# Autodesk Inventor assembly: R-H v20
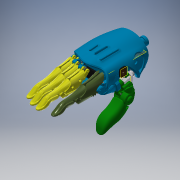
[picture p0: Inventor's stored thumbnail of the model, 180x180]
Saved by Autodesk Inventor 2018.2 (Build 222227000, 227)
## iProperties
Created: 2017-09-22
Part Number: R-H v20
Material: 一般
Document SubType Name: Assembly
Designer: sktom
Author: sktom
## Documents named in this file (41)
- D:\CloudStrage\OneDrive\CADMech\HbSizeMMech\UnitHand\Unit_MR-H\Unit_MR-H.iam
- D:\CloudStrage\OneDrive\CADMech\HbSizeMMech\UnitHand\Unit_MR-H\Parts_MR-H\MR-H-01.ipt
- D:\CloudStrage\OneDrive\CADMech\HbSizeMMech\UnitHand\Unit_MR-H\Parts_MR-H\MR-H-02.ipt
- D:\CloudStrage\OneDrive\CADMech\HbSizeMMech\UnitHand\Unit_MR-H\Parts_MR-H\MR-H-03.ipt
- D:\CloudStrage\OneDrive\CADMech\HbSizeMMech\UnitHand\Unit_MR-H\Parts_MR-H\MR-H-04.ipt
- D:\CloudStrage\OneDrive\CADMech\HbSizeMMech\UnitHand\Unit_MR-H\Unit_MR-I\Unit_MR-I .iam
- D:\CloudStrage\OneDrive\CADMech\HbSizeMMech\UnitHand\Unit_MR-H\Unit_MR-O\Unit_MR-O.iam
- D:\CloudStrage\OneDrive\CADMech\HbSizeMMech\UnitHand\Unit_MR-H\Parts_MR-H\MR-H-05.ipt
- D:\CloudStrage\OneDrive\CADMech\HbSizeMMech\UnitHand\Unit_MR-H\Parts_MR-H\MR-H-06.ipt
- D:\CloudStrage\OneDrive\CADMech\HbSizeMMech\UnitHand\Unit_MR-H\Parts_MR-H\MR-H-07.ipt
- D:\CloudStrage\OneDrive\CADMech\HbSizeMMech\UnitHand\Unit_MR-H\Parts_MR-H\MR-H-08.ipt
- D:\CloudStrage\OneDrive\CADMech\HbSizeMMech\UnitHand\Unit_MR-H\Parts_MR-H\MR-H-15.ipt
- D:\CloudStrage\OneDrive\CADMech\HbSizeMMech\UnitHand\Unit_MR-H\Parts_MR-H\MR-H-10.ipt
- D:\CloudStrage\OneDrive\CADMech\HbSizeMMech\UnitHand\Unit_MR-H\Parts_MR-H\MR-H-11.ipt
- D:\CloudStrage\OneDrive\CADMech\HbSizeMMech\UnitHand\Unit_MR-H\Parts_MR-H\MR-H-12.ipt
- D:\CloudStrage\OneDrive\CADMech\HbSizeMMech\UnitHand\Unit_MR-H\Parts_MR-H\MR-H-13.ipt
- D:\CloudStrage\OneDrive\CADMech\HbSizeMMech\UnitHand\Unit_MR-H\Parts_MR-H\MR-H-14.ipt
- D:\CloudStrage\OneDrive\CADMech\HbSizeMMech\UnitHand\Unit_MR-H\Unit_MR-T\Unit_MR-T.iam
- D:\CloudStrage\OneDrive\CADMech\HbSizeMMech\UnitHand\Unit_MR-H\Parts_MR-H\Parts_bearing_FL674ZZ.ipt
- D:\CloudStrage\OneDrive\CADMech\HbSizeMMech\UnitHand\Unit_MR-H\Parts_MR-H\Parts_Servo_Micro2BBMG.ipt
- D:\CloudStrage\OneDrive\CADMech\HbSizeMMech\UnitHand\Unit_MR-H\Parts_MR-H\Parts_Servo_HK282A_Hone.ipt
- D:\CloudStrage\OneDrive\CADMech\HbSizeMMech\UnitHand\Unit_MR-H\Parts_MR-H\Parts_Servo_ASV-15MG.ipt
- D:\CloudStrage\OneDrive\CADMech\HbSizeMMech\UnitHand\Unit_MR-H\Parts_MR-H\MR-H-09.ipt
- D:\CloudStrage\OneDrive\CADMech\HbSizeMMech\UnitHand\Unit_MR-H\Parts_MR-H\Circuit_handmainboard.ipt
- D:\CloudStrage\OneDrive\CADMech\HbSizeMMech\UnitHand\Unit_MR-H\Parts_MR-H\Parts_Screw_M1.7_L8.ipt
- D:\CloudStrage\OneDrive\CADMech\HbSizeMMech\UnitHand\Unit_MR-H\Parts_MR-H\Parts_Screw_M2_L8.ipt
- D:\CloudStrage\OneDrive\CADMech\HbSizeMMech\UnitHand\Unit_MR-H\Parts_MR-H\Parts_Screw_M3_L6.ipt
- D:\CloudStrage\OneDrive\CADMech\HbSizeMMech\UnitHand\Unit_MR-H\Parts_MR-H\Parts_Servo_Micro2BBMG_hone.ipt
- D:\CloudStrage\OneDrive\CADMech\HbSizeMMech\UnitHand\Unit_MR-H\Parts_MR-H\Parts_FlatScrew_M2_L6.ipt
- D:\CloudStrage\OneDrive\CADMech\HbSizeMMech\UnitHand\Unit_MR-H\Parts_MR-H\Parts_Shaft_Phi2_L12.ipt
- D:\CloudStrage\OneDrive\CADMech\HbSizeMMech\UnitHand\Unit_MR-H\Parts_MR-H\Parts_MetalCollar_Ph2_L4.5.ipt
- D:\CloudStrage\OneDrive\CADMech\HbSizeMMech\UnitHand\Unit_MR-H\Parts_MR-H\Parts_Washer_M2_Ph4.3_T0.3.ipt
- D:\CloudStrage\OneDrive\CADMech\HbSizeMMech\UnitHand\Unit_MR-H\Parts_MR-H\Parts_Servo_ASV-15MG_Hone.ipt
- D:\CloudStrage\OneDrive\CADMech\HbSizeMMech\UnitHand\Unit_MR-H\Parts_MR-H\Circuit_Controller_Pololu-A-Star-32U4-Micro.ipt
- D:\CloudStrage\OneDrive\CADMech\HbSizeMMech\UnitHand\Unit_MR-H\Parts_MR-H\Circuit_DCDCconverter_OKL-T3-W12N-C.ipt
- D:\CloudStrage\OneDrive\CADMech\HbSizeMMech\UnitHand\Unit_MR-H\Parts_MR-H\Circuit_DCjack_MJ179PH.ipt
- D:\CloudStrage\OneDrive\CADMech\HbSizeMMech\UnitHand\Unit_MR-H\Parts_MR-H\Circuit_Connector_533980371.ipt
- D:\CloudStrage\OneDrive\CADMech\HbSizeMMech\UnitHand\Unit_MR-H\Parts_MR-H\Circuit_Connector_H3-2.ipt
- D:\CloudStrage\OneDrive\CADMech\HbSizeMMech\UnitHand\Unit_MR-H\Parts_MR-H\Circuit_TactSwitch_SKRPACE010.ipt
- D:\CloudStrage\OneDrive\CADMech\HbSizeMMech\UnitHand\Unit_MR-H\Parts_MR-H\Circuit_SlideSwitch_SS-12D00-G5.ipt
- D:\CloudStrage\OneDrive\CADMech\HbSizeMMech\UnitHand\Unit_MR-H\Parts_MR-H\Circuit_PinHeader_PSM-410233-00.ipt
## Components (89 placed, 40 different names)
1. Unit_MR-I [sub-assembly] — メイト:25, 円柱状:15
2. Unit_MR-T:1 [sub-assembly]
3. Unit_MR-O:2 [sub-assembly] — 挿入:42, 円柱状:5, 円柱状:6, メイト:22, 挿入:43
4. Unit_MR-O:4 [sub-assembly] — メイト:24, 円柱状:12, 円柱状:13, 挿入:54, 挿入:55, 挿入:56
5. Unit_MR-O:3 [sub-assembly] — メイト:23, 円柱状:8, 円柱状:9, 挿入:46, 挿入:49, 挿入:50, 挿入:51
6. MR-H-01:1
7. MR-H-02:1 — 挿入:1, 挿入:2, 挿入:13, 挿入:14, 挿入:17, 挿入:18, 挿入:22, 挿入:26, 挿入:32, 挿入:33, 円柱状:5, 円柱状:6, メイト:22, メイト:23, 円柱状:8, 円柱状:9, メイト:24, 円柱状:12, 円柱状:13, メイト:25, 円柱状:15, 挿入:59, 挿入:60, 円柱状:16, 挿入:61, 円柱状:17, 挿入:62, 円柱状:18, 挿入:63, 挿入:64, 挿入:65, 挿入:66, 挿入:67, 円柱状:19, メイト:30
8. MR-H-03:1 — 挿入:26, 挿入:27
9. MR-H-04:1 — 挿入:22, 挿入:23
10. MR-H-05:1 — 円柱状:7, 円柱状:10
11. MR-H-06:1 — 円柱状:11, 円柱状:14
12. MR-H-07:1 — 円柱状:4, 回転:3
13. MR-H-08:1 — 挿入:20, 挿入:21, 回転:1, 回転:2
14. MR-H-09:1 — 挿入:28, 挿入:29, 挿入:30, 挿入:31, 挿入:32, 挿入:33, 挿入:34, 挿入:35, 挿入:36, 挿入:37
15. MR-H-10:1 — フラッシュ:1, フラッシュ:3, メイト:4, フラッシュ:5
16. MR-H-11:1 — フラッシュ:1, フラッシュ:2, フラッシュ:3, フラッシュ:4, メイト:4, メイト:5
17. MR-H-12:1 — フラッシュ:2, フラッシュ:4, メイト:5
18. MR-H-13:1 — 円柱状:1, 円柱状:2, メイト:9, フラッシュ:5
19. MR-H-14:1 — メイト:2, 円柱状:3, メイト:7
20. MR-H-15:1 — 円柱状:1, 円柱状:2, メイト:2, 円柱状:3, メイト:9, 挿入:1, 挿入:2, 挿入:15, 挿入:16, 挿入:68, フラッシュ:17, 挿入:69, 挿入:70, 挿入:71, 挿入:72
21. Parts_Screw_M1.7_L8:1 — 挿入:23
22. Parts_Screw_M1.7_L8:2 — 挿入:27
23. Parts_Screw_M1.7_L8:3 — 挿入:12
24. Parts_Screw_M1.7_L8:4 — 挿入:11
25. Parts_Screw_M1.7_L8:5 — 挿入:16
26. Parts_Screw_M1.7_L8:6 — 挿入:15
27. Parts_Screw_M1.7_L8:7 — 挿入:67
28. Parts_Screw_M1.7_L8:8 — 挿入:66
29. Parts_Screw_M1.7_L8:9 — 挿入:68
30. Parts_Screw_M2_L8:3 — 挿入:55
31. Parts_Screw_M2_L8:4 — 挿入:50
32. Parts_Screw_M2_L8:5
33. Parts_Screw_M2_L8:6 — 挿入:41
34. Parts_Screw_M2_L8:7 — 挿入:45
35. Parts_Screw_M2_L8:8 — 挿入:48
36. Parts_Screw_M2_L8:9 — 挿入:53
37. Parts_Screw_M2_L8:10 — 挿入:58
38. Parts_Screw_M2_L8:11 — 挿入:30
39. Parts_Screw_M2_L8:12 — 挿入:31
40. Parts_Screw_M2_L8:13 — 挿入:64
41. Parts_Screw_M2_L8:14 — 挿入:63
42. Parts_FlatScrew_M2_L6:1 — 回転:1
43. Parts_FlatScrew_M2_L6:2 — 回転:2
44. Parts_FlatScrew_M2_L6:3 — 挿入:34
45. Parts_FlatScrew_M2_L6:4 — 挿入:37
46. Parts_FlatScrew_M2_L6:5 — 挿入:36
47. Parts_FlatScrew_M2_L6:6 — 挿入:35
48. Parts_Screw_M3_L6:1 — 挿入:24
49. Parts_Screw_M3_L6:2 — 挿入:25
50. Parts_Shaft_Phi2_L12:1 — 挿入:59
51. Parts_Shaft_Phi2_L12:2 — 挿入:60, フラッシュ:13
52. Parts_Shaft_Phi2_L12:3 — フラッシュ:13, 円柱状:16
53. Parts_Shaft_Phi2_L12:4 — 挿入:61, フラッシュ:14
54. Parts_Shaft_Phi2_L12:5 — フラッシュ:14, 円柱状:17
55. Parts_Shaft_Phi2_L12:6 — 挿入:62, フラッシュ:15
56. Parts_Shaft_Phi2_L12:7 — フラッシュ:15, 円柱状:18
57. Parts_MetalCollar_Ph2_L4.5:1 — 挿入:56, 挿入:57, 円柱状:14
58. Parts_MetalCollar_Ph2_L4.5:2 — 挿入:51, 挿入:52, 円柱状:11
59. Parts_MetalCollar_Ph2_L4.5:3 — 挿入:46, 挿入:47, 円柱状:10
60. Parts_MetalCollar_Ph2_L4.5:4 — 挿入:43, 挿入:44, 円柱状:7
61. Parts_MetalCollar_Ph2_L4.5:5 — 挿入:54
62. Parts_MetalCollar_Ph2_L4.5:6 — 挿入:39, 挿入:40, 円柱状:4
63. Parts_MetalCollar_Ph2_L4.5:7 — 挿入:49
64. Parts_MetalCollar_Ph2_L4.5:8 — 挿入:42, 回転:3
65. Parts_Washer_M2_Ph4.3_T0.3:1 — 挿入:44, 挿入:45
66. Parts_Washer_M2_Ph4.3_T0.3:2 — 挿入:57, 挿入:58
67. Parts_Washer_M2_Ph4.3_T0.3:3 — 挿入:47, 挿入:48
68. Parts_Washer_M2_Ph4.3_T0.3:4 — 挿入:52, 挿入:53
69. Parts_Washer_M2_Ph4.3_T0.3:5 — 挿入:40, 挿入:41
70. Parts_Servo_HK282A_Hone:1 — 挿入:11, 挿入:12, 挿入:13, 挿入:14
71. Parts_Servo_ASV-15MG:1 — 挿入:28, 挿入:29, 挿入:38
72. Parts_Servo_ASV-15MG_Hone:1 — 挿入:38, 挿入:39
73. Parts_Servo_Micro2BBMG:1 — 挿入:17, 挿入:18, 挿入:19, 挿入:24, 挿入:25
74. Parts_Servo_Micro2BBMG_hone:1 — 挿入:19, 挿入:20, 挿入:21
75. Parts_bearing_FL674ZZ:1 — 挿入:65
76. Circuit_handmainboard:1 — メイト:11, メイト:12, メイト:13, メイト:14, メイト:17, メイト:18, メイト:19, メイト:20, メイト:26, フラッシュ:16, フラッシュ:17, 挿入:69, 挿入:70, 挿入:71, 挿入:72, フラッシュ:18, フラッシュ:19, メイト:27, フラッシュ:21, フラッシュ:22, メイト:29
77. Circuit_Controller_Pololu-A-Star-32U4-Micro:1 — 挿入:7, 挿入:8, 挿入:9, 挿入:10, フラッシュ:18
78. Circuit_DCDCconverter_OKL-T3-W12N-C:1 — メイト:17
79. Circuit_DCjack_MJ179PH:1 — 円柱状:19, メイト:29, メイト:30
80. Circuit_PinHeader_PSM-410233-00:1 — 挿入:7, 挿入:8, メイト:18
81. Circuit_PinHeader_PSM-410233-00:2 — 挿入:9, 挿入:10, フラッシュ:19
82. Circuit_Connector_533980371:1 — メイト:26, フラッシュ:16, メイト:27, メイト:28, フラッシュ:20
83. Circuit_Connector_H3-2:1 — メイト:20, フラッシュ:21, フラッシュ:22
84. Circuit_Connector_H3-2:2 — メイト:19, メイト:28, フラッシュ:20
85. Circuit_SlideSwitch_SS-12D00-G5:1 — メイト:7
86. Circuit_TactSwitch_SKRPACE010:1 — メイト:11, フラッシュ:8
87. Circuit_TactSwitch_SKRPACE010:2 — メイト:12, フラッシュ:7, フラッシュ:8
88. Circuit_TactSwitch_SKRPACE010:3 — メイト:13, フラッシュ:7
89. Circuit_TactSwitch_SKRPACE010:4 — メイト:14
## Relationships (129: Insert 68, Mate 22, CylindricalJoint 19, Flush 17, RevoluteJoint 3)
- 円柱状:1 [CylindricalJoint]: MR-H-13:1 ↔ MR-H-15:1
- 円柱状:2 [CylindricalJoint]: MR-H-13:1 ↔ MR-H-15:1
- メイト:2 [Mate] (0.2 mm): MR-H-14:1 ↔ MR-H-15:1
- 円柱状:3 [CylindricalJoint]: MR-H-14:1 ↔ MR-H-15:1
- フラッシュ:1 [Flush]: MR-H-10:1 ↔ MR-H-11:1
- フラッシュ:2 [Flush]: MR-H-11:1 ↔ MR-H-12:1
- フラッシュ:3 [Flush]: MR-H-10:1 ↔ MR-H-11:1
- フラッシュ:4 [Flush]: MR-H-11:1 ↔ MR-H-12:1
- メイト:4 [Mate] (0.2 mm): MR-H-10:1 ↔ MR-H-11:1
- メイト:5 [Mate] (0.2 mm): MR-H-11:1 ↔ MR-H-12:1
- メイト:7 [Mate] (0.2 mm): MR-H-14:1 ↔ Circuit_SlideSwitch_SS-12D00-G5:1
- メイト:9 [Mate] (0.2 mm): MR-H-13:1 ↔ MR-H-15:1
- フラッシュ:5 [Flush]: MR-H-10:1 ↔ MR-H-13:1
- 挿入:1 [Insert]: MR-H-02:1 ↔ MR-H-15:1
- 挿入:2 [Insert]: MR-H-02:1 ↔ MR-H-15:1
- メイト:11 [Mate]: Circuit_handmainboard:1 ↔ Circuit_TactSwitch_SKRPACE010:1
- メイト:12 [Mate]: Circuit_handmainboard:1 ↔ Circuit_TactSwitch_SKRPACE010:2
- メイト:13 [Mate]: Circuit_handmainboard:1 ↔ Circuit_TactSwitch_SKRPACE010:3
- フラッシュ:7 [Flush]: Circuit_TactSwitch_SKRPACE010:2 ↔ Circuit_TactSwitch_SKRPACE010:3
- フラッシュ:8 [Flush]: Circuit_TactSwitch_SKRPACE010:1 ↔ Circuit_TactSwitch_SKRPACE010:2
- メイト:14 [Mate]: Circuit_handmainboard:1 ↔ Circuit_TactSwitch_SKRPACE010:4
- メイト:17 [Mate]: Circuit_handmainboard:1 ↔ Circuit_DCDCconverter_OKL-T3-W12N-C:1
- 挿入:7 [Insert]: Circuit_Controller_Pololu-A-Star-32U4-Micro:1 ↔ Circuit_PinHeader_PSM-410233-00:1
- 挿入:8 [Insert]: Circuit_Controller_Pololu-A-Star-32U4-Micro:1 ↔ Circuit_PinHeader_PSM-410233-00:1
- 挿入:9 [Insert]: Circuit_Controller_Pololu-A-Star-32U4-Micro:1 ↔ Circuit_PinHeader_PSM-410233-00:2
- 挿入:10 [Insert]: Circuit_Controller_Pololu-A-Star-32U4-Micro:1 ↔ Circuit_PinHeader_PSM-410233-00:2
- メイト:18 [Mate]: Circuit_handmainboard:1 ↔ Circuit_PinHeader_PSM-410233-00:1
- メイト:19 [Mate]: Circuit_handmainboard:1 ↔ Circuit_Connector_H3-2:2
- メイト:20 [Mate]: Circuit_handmainboard:1 ↔ Circuit_Connector_H3-2:1
- 挿入:11 [Insert]: Parts_Screw_M1.7_L8:4 ↔ Parts_Servo_HK282A_Hone:1
- 挿入:12 [Insert]: Parts_Screw_M1.7_L8:3 ↔ Parts_Servo_HK282A_Hone:1
- 挿入:13 [Insert]: MR-H-02:1 ↔ Parts_Servo_HK282A_Hone:1
- 挿入:14 [Insert]: MR-H-02:1 ↔ Parts_Servo_HK282A_Hone:1
- 挿入:15 [Insert]: MR-H-15:1 ↔ Parts_Screw_M1.7_L8:6
- 挿入:16 [Insert]: MR-H-15:1 ↔ Parts_Screw_M1.7_L8:5
- 挿入:17 [Insert]: MR-H-02:1 ↔ Parts_Servo_Micro2BBMG:1
- 挿入:18 [Insert]: MR-H-02:1 ↔ Parts_Servo_Micro2BBMG:1
- 挿入:19 [Insert]: Parts_Servo_Micro2BBMG:1 ↔ Parts_Servo_Micro2BBMG_hone:1
- 挿入:20 [Insert]: MR-H-08:1 ↔ Parts_Servo_Micro2BBMG_hone:1
- 挿入:21 [Insert]: MR-H-08:1 ↔ Parts_Servo_Micro2BBMG_hone:1
- 挿入:22 [Insert]: MR-H-02:1 ↔ MR-H-04:1
- 挿入:23 [Insert]: MR-H-04:1 ↔ Parts_Screw_M1.7_L8:1
- 挿入:24 [Insert]: Parts_Screw_M3_L6:1 ↔ Parts_Servo_Micro2BBMG:1
- 挿入:25 [Insert]: Parts_Screw_M3_L6:2 ↔ Parts_Servo_Micro2BBMG:1
- 回転:1 [RevoluteJoint]: MR-H-08:1 ↔ Parts_FlatScrew_M2_L6:1
- 回転:2 [RevoluteJoint]: MR-H-08:1 ↔ Parts_FlatScrew_M2_L6:2
- 挿入:26 [Insert]: MR-H-02:1 ↔ MR-H-03:1
- 挿入:27 [Insert]: MR-H-03:1 ↔ Parts_Screw_M1.7_L8:2
- 挿入:28 [Insert]: MR-H-09:1 ↔ Parts_Servo_ASV-15MG:1
- 挿入:29 [Insert]: MR-H-09:1 ↔ Parts_Servo_ASV-15MG:1
- 挿入:30 [Insert]: MR-H-09:1 ↔ Parts_Screw_M2_L8:11
- 挿入:31 [Insert]: MR-H-09:1 ↔ Parts_Screw_M2_L8:12
- 挿入:32 [Insert]: MR-H-02:1 ↔ MR-H-09:1
- 挿入:33 [Insert]: MR-H-02:1 ↔ MR-H-09:1
- 挿入:34 [Insert]: MR-H-09:1 ↔ Parts_FlatScrew_M2_L6:3
- 挿入:35 [Insert]: MR-H-09:1 ↔ Parts_FlatScrew_M2_L6:6
- 挿入:36 [Insert]: MR-H-09:1 ↔ Parts_FlatScrew_M2_L6:5
- 挿入:37 [Insert]: MR-H-09:1 ↔ Parts_FlatScrew_M2_L6:4
- 挿入:38 [Insert]: Parts_Servo_ASV-15MG:1 ↔ Parts_Servo_ASV-15MG_Hone:1
- 挿入:39 [Insert]: Parts_MetalCollar_Ph2_L4.5:6 ↔ Parts_Servo_ASV-15MG_Hone:1
- 挿入:40 [Insert]: Parts_MetalCollar_Ph2_L4.5:6 ↔ Parts_Washer_M2_Ph4.3_T0.3:5
- 挿入:41 [Insert]: Parts_Screw_M2_L8:6 ↔ Parts_Washer_M2_Ph4.3_T0.3:5
- 円柱状:4 [CylindricalJoint]: MR-H-07:1 ↔ Parts_MetalCollar_Ph2_L4.5:6
- 挿入:42 [Insert]: Unit_MR-O:2 ↔ Parts_MetalCollar_Ph2_L4.5:8
- 円柱状:5 [CylindricalJoint]: Unit_MR-O:2 ↔ MR-H-02:1
- 円柱状:6 [CylindricalJoint]: Unit_MR-O:2 ↔ MR-H-02:1
- メイト:22 [Mate] (0.1 mm): Unit_MR-O:2 ↔ MR-H-02:1
- 回転:3 [RevoluteJoint]: MR-H-07:1 ↔ Parts_MetalCollar_Ph2_L4.5:8
- 挿入:43 [Insert]: Unit_MR-O:2 ↔ Parts_MetalCollar_Ph2_L4.5:4
- 挿入:44 [Insert]: Parts_MetalCollar_Ph2_L4.5:4 ↔ Parts_Washer_M2_Ph4.3_T0.3:1
- 挿入:45 [Insert]: Parts_Screw_M2_L8:7 ↔ Parts_Washer_M2_Ph4.3_T0.3:1
- 円柱状:7 [CylindricalJoint]: MR-H-05:1 ↔ Parts_MetalCollar_Ph2_L4.5:4
- メイト:23 [Mate] (0.1 mm): Unit_MR-O:3 ↔ MR-H-02:1
- 円柱状:8 [CylindricalJoint]: Unit_MR-O:3 ↔ MR-H-02:1
- 円柱状:9 [CylindricalJoint]: Unit_MR-O:3 ↔ MR-H-02:1
- 挿入:46 [Insert]: Unit_MR-O:3 ↔ Parts_MetalCollar_Ph2_L4.5:3
- 挿入:47 [Insert]: Parts_MetalCollar_Ph2_L4.5:3 ↔ Parts_Washer_M2_Ph4.3_T0.3:3
- 挿入:48 [Insert]: Parts_Screw_M2_L8:8 ↔ Parts_Washer_M2_Ph4.3_T0.3:3
- 円柱状:10 [CylindricalJoint]: MR-H-05:1 ↔ Parts_MetalCollar_Ph2_L4.5:3
- 挿入:49 [Insert]: Unit_MR-O:3 ↔ Parts_MetalCollar_Ph2_L4.5:7
- 挿入:50 [Insert]: Unit_MR-O:3 ↔ Parts_Screw_M2_L8:4
- 挿入:51 [Insert]: Unit_MR-O:3 ↔ Parts_MetalCollar_Ph2_L4.5:2
- 挿入:52 [Insert]: Parts_MetalCollar_Ph2_L4.5:2 ↔ Parts_Washer_M2_Ph4.3_T0.3:4
- 挿入:53 [Insert]: Parts_Screw_M2_L8:9 ↔ Parts_Washer_M2_Ph4.3_T0.3:4
- 円柱状:11 [CylindricalJoint]: MR-H-06:1 ↔ Parts_MetalCollar_Ph2_L4.5:2
- メイト:24 [Mate] (0.1 mm): Unit_MR-O:4 ↔ MR-H-02:1
- 円柱状:12 [CylindricalJoint]: Unit_MR-O:4 ↔ MR-H-02:1
- 円柱状:13 [CylindricalJoint]: Unit_MR-O:4 ↔ MR-H-02:1
- 挿入:54 [Insert]: Unit_MR-O:4 ↔ Parts_MetalCollar_Ph2_L4.5:5
- 挿入:55 [Insert]: Unit_MR-O:4 ↔ Parts_Screw_M2_L8:3
- 挿入:56 [Insert]: Unit_MR-O:4 ↔ Parts_MetalCollar_Ph2_L4.5:1
- 挿入:57 [Insert]: Parts_MetalCollar_Ph2_L4.5:1 ↔ Parts_Washer_M2_Ph4.3_T0.3:2
- 挿入:58 [Insert]: Parts_Screw_M2_L8:10 ↔ Parts_Washer_M2_Ph4.3_T0.3:2
- 円柱状:14 [CylindricalJoint]: MR-H-06:1 ↔ Parts_MetalCollar_Ph2_L4.5:1
- メイト:25 [Mate] (0.184 mm): Unit_MR-I ↔ MR-H-02:1
- 円柱状:15 [CylindricalJoint]: Unit_MR-I ↔ MR-H-02:1
- 挿入:59 [Insert] (1 mm): MR-H-02:1 ↔ Parts_Shaft_Phi2_L12:1
- 挿入:60 [Insert] (0.4 mm): MR-H-02:1 ↔ Parts_Shaft_Phi2_L12:2
- フラッシュ:13 [Flush]: Parts_Shaft_Phi2_L12:2 ↔ Parts_Shaft_Phi2_L12:3
- 円柱状:16 [CylindricalJoint]: MR-H-02:1 ↔ Parts_Shaft_Phi2_L12:3
- 挿入:61 [Insert] (0.4 mm): MR-H-02:1 ↔ Parts_Shaft_Phi2_L12:4
- フラッシュ:14 [Flush]: Parts_Shaft_Phi2_L12:4 ↔ Parts_Shaft_Phi2_L12:5
- 円柱状:17 [CylindricalJoint]: MR-H-02:1 ↔ Parts_Shaft_Phi2_L12:5
- 挿入:62 [Insert] (0.4 mm): MR-H-02:1 ↔ Parts_Shaft_Phi2_L12:6
- フラッシュ:15 [Flush]: Parts_Shaft_Phi2_L12:6 ↔ Parts_Shaft_Phi2_L12:7
- 円柱状:18 [CylindricalJoint]: MR-H-02:1 ↔ Parts_Shaft_Phi2_L12:7
- 挿入:63 [Insert]: MR-H-02:1 ↔ Parts_Screw_M2_L8:14
- 挿入:64 [Insert]: MR-H-02:1 ↔ Parts_Screw_M2_L8:13
- 挿入:65 [Insert]: MR-H-02:1 ↔ Parts_bearing_FL674ZZ:1
- 挿入:66 [Insert]: MR-H-02:1 ↔ Parts_Screw_M1.7_L8:8
- 挿入:67 [Insert]: MR-H-02:1 ↔ Parts_Screw_M1.7_L8:7
- 挿入:68 [Insert]: MR-H-15:1 ↔ Parts_Screw_M1.7_L8:9
- メイト:26 [Mate]: Circuit_handmainboard:1 ↔ Circuit_Connector_533980371:1
- フラッシュ:16 [Flush] (1 mm): Circuit_handmainboard:1 ↔ Circuit_Connector_533980371:1
- フラッシュ:17 [Flush]: MR-H-15:1 ↔ Circuit_handmainboard:1
- 挿入:69 [Insert]: MR-H-15:1 ↔ Circuit_handmainboard:1
- 挿入:70 [Insert]: MR-H-15:1 ↔ Circuit_handmainboard:1
- 挿入:71 [Insert]: MR-H-15:1 ↔ Circuit_handmainboard:1
- 挿入:72 [Insert]: MR-H-15:1 ↔ Circuit_handmainboard:1
- フラッシュ:18 [Flush]: Circuit_handmainboard:1 ↔ Circuit_Controller_Pololu-A-Star-32U4-Micro:1
- フラッシュ:19 [Flush] (-9 mm): Circuit_handmainboard:1 ↔ Circuit_PinHeader_PSM-410233-00:2
- メイト:27 [Mate] (4 mm): Circuit_handmainboard:1 ↔ Circuit_Connector_533980371:1
- メイト:28 [Mate] (2 mm): Circuit_Connector_533980371:1 ↔ Circuit_Connector_H3-2:2
- フラッシュ:20 [Flush]: Circuit_Connector_533980371:1 ↔ Circuit_Connector_H3-2:2
- フラッシュ:21 [Flush] (-1 mm): Circuit_handmainboard:1 ↔ Circuit_Connector_H3-2:1
- フラッシュ:22 [Flush] (8.5 mm): Circuit_handmainboard:1 ↔ Circuit_Connector_H3-2:1
- 円柱状:19 [CylindricalJoint]: MR-H-02:1 ↔ Circuit_DCjack_MJ179PH:1
- メイト:29 [Mate]: Circuit_handmainboard:1 ↔ Circuit_DCjack_MJ179PH:1
- メイト:30 [Mate] (0.5 mm): MR-H-02:1 ↔ Circuit_DCjack_MJ179PH:1
